# Autodesk Inventor assembly: HandRight
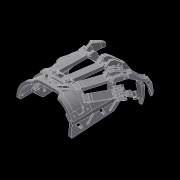
[picture p0: Inventor's stored thumbnail of the model, 180x180]
Saved by Autodesk Inventor 2015 SP1 (Build 190203100, 203)
## iProperties
Created: 2014-12-21
Part Number: HandRight
Document SubType Name: Assembly
Designer: Inventor
Mass: 48.1874 g
Surface Area: 412.068 cm^2
Volume: 48.1874 cm^3
Density: 1 g/cm^3
Author: Inventor
## Documents named in this file (22)
- E:\Exo\Models\3D\HandRight.iam
- E:\Exo\Models\3D\HandShockPlateRight.ipt
- E:\Exo\Models\3D\ThumbShockPlateRight.ipt
- E:\Exo\Models\3D\HandRibRight.ipt
- E:\Exo\Models\3D\ThumbMount.ipt
- E:\Exo\Models\3D\MetacarpusIndex.ipt
- E:\Exo\Models\3D\MetacarpusMiddle.ipt
- E:\Exo\Models\3D\MetacarpusRing.ipt
- E:\Exo\Models\3D\MetacarpusPinky.ipt
- E:\Exo\Models\3D\MetacarpusThumb.ipt
- E:\Exo\Models\3D\ProxPhalangeIndex.ipt
- E:\Exo\Models\3D\ProxPhalangeMiddle.ipt
- E:\Exo\Models\3D\ProxPhalangePinky.ipt
- E:\Exo\Models\3D\ProxPhalangeRing.ipt
- E:\Exo\Models\3D\ProxPhalangeThumb.ipt
- E:\Exo\Models\3D\Knuckle.ipt
- E:\Exo\Models\3D\KnuckleSide.ipt
- E:\Exo\Models\3D\DistPhalangeIndex.ipt
- E:\Exo\Models\3D\DistPhalangeMiddle.ipt
- E:\Exo\Models\3D\DistPhalangePinky.ipt
- E:\Exo\Models\3D\DistPhalangeRing.ipt
- E:\Exo\Models\3D\DistPhalangeThumb.ipt
## Components (34 placed, 21 different names)
1. HandShockPlateRight:1 — Mate:2, Mate:4, Mate:5, Mate:11, Mate:12, Mate:13, Mate:14
2. ThumbShockPlateRight:1 — Mate:4, Mate:5, Mate:6, Mate:7, Mate:10
3. HandRibRight:1 — Mate:2
4. ThumbMount:1 — Mate:6, Mate:7, Mate:8, Mate:9, Mate:10
5. MetacarpusIndex:1 — Mate:11, Mate:20, Mate:21, Mate:42, Mate:44, Mate:46
6. MetacarpusMiddle:1 — Mate:12, Mate:22, Mate:23, Mate:48, Mate:49, Mate:51, Mate:52
7. MetacarpusRing:1 — Mate:13, Mate:24, Mate:25, Mate:54, Mate:55, Mate:57, Mate:58
8. MetacarpusPinky:1 — Mate:14, Mate:26, Mate:27, Mate:60, Mate:61, Mate:63, Mate:64
9. MetacarpusThumb:1 — Mate:8, Mate:9, Mate:16, Mate:17, Mate:36, Mate:39
10. ProxPhalangeIndex:1 — Mate:28, Mate:29, Mate:43, Mate:45, Mate:47, Mate:66
11. ProxPhalangeMiddle:1 — Mate:30, Mate:31, Mate:50, Mate:53, Mate:67
12. ProxPhalangePinky:1 — Mate:34, Mate:35, Mate:62, Mate:65, Mate:69
13. ProxPhalangeRing:1 — Mate:32, Mate:33, Mate:56, Mate:59, Mate:68
14. ProxPhalangeThumb:1 — Mate:18, Mate:19, Mate:37, Mate:38, Mate:40, Mate:41, Mate:70
15. Knuckle:1 — Mate:26, Mate:27, Mate:34, Mate:35
16. Knuckle:2 — Mate:24, Mate:25, Mate:32, Mate:33
17. Knuckle:3 — Mate:22, Mate:23, Mate:30, Mate:31
18. Knuckle:4 — Mate:20, Mate:21, Mate:28, Mate:29
19. Knuckle:5 — Mate:16, Mate:17, Mate:18, Mate:19
20. KnuckleSide:1 — Mate:36, Mate:37, Mate:38
21. KnuckleSide:2 — Mate:39, Mate:40, Mate:41
22. KnuckleSide:3 — Mate:42, Mate:43, Mate:44
23. KnuckleSide:4 — Mate:45, Mate:46, Mate:47
24. KnuckleSide:5 — Mate:48, Mate:49, Mate:50
25. KnuckleSide:6 — Mate:51, Mate:52, Mate:53
26. KnuckleSide:7 — Mate:54, Mate:55, Mate:56
27. KnuckleSide:8 — Mate:57, Mate:58, Mate:59
28. KnuckleSide:9 — Mate:63, Mate:64, Mate:65
29. KnuckleSide:10 — Mate:60, Mate:61, Mate:62
30. DistPhalangeIndex:1 — Mate:66
31. DistPhalangeMiddle:1 — Mate:67
32. DistPhalangePinky:1 — Mate:69
33. DistPhalangeRing:1 — Mate:68
34. DistPhalangeThumb:1 — Mate:70
## Relationships (67: Mate 67)
- Mate:2: HandShockPlateRight:1 ↔ HandRibRight:1
- Mate:4: HandShockPlateRight:1 ↔ ThumbShockPlateRight:1
- Mate:5: HandShockPlateRight:1 ↔ ThumbShockPlateRight:1
- Mate:6: ThumbShockPlateRight:1 ↔ ThumbMount:1
- Mate:7: ThumbShockPlateRight:1 ↔ ThumbMount:1
- Mate:8: ThumbMount:1 ↔ MetacarpusThumb:1
- Mate:9: ThumbMount:1 ↔ MetacarpusThumb:1
- Mate:10: ThumbShockPlateRight:1 ↔ ThumbMount:1
- Mate:11: HandShockPlateRight:1 ↔ MetacarpusIndex:1
- Mate:12: HandShockPlateRight:1 ↔ MetacarpusMiddle:1
- Mate:13: HandShockPlateRight:1 ↔ MetacarpusRing:1
- Mate:14: HandShockPlateRight:1 ↔ MetacarpusPinky:1
- Mate:16: MetacarpusThumb:1 ↔ Knuckle:5
- Mate:17: MetacarpusThumb:1 ↔ Knuckle:5
- Mate:18: ProxPhalangeThumb:1 ↔ Knuckle:5
- Mate:19: ProxPhalangeThumb:1 ↔ Knuckle:5
- Mate:20: MetacarpusIndex:1 ↔ Knuckle:4
- Mate:21: MetacarpusIndex:1 ↔ Knuckle:4
- Mate:22: MetacarpusMiddle:1 ↔ Knuckle:3
- Mate:23: MetacarpusMiddle:1 ↔ Knuckle:3
- Mate:24: MetacarpusRing:1 ↔ Knuckle:2
- Mate:25: MetacarpusRing:1 ↔ Knuckle:2
- Mate:26: MetacarpusPinky:1 ↔ Knuckle:1
- Mate:27: MetacarpusPinky:1 ↔ Knuckle:1
- Mate:28: ProxPhalangeIndex:1 ↔ Knuckle:4
- Mate:29: ProxPhalangeIndex:1 ↔ Knuckle:4
- Mate:30: ProxPhalangeMiddle:1 ↔ Knuckle:3
- Mate:31: ProxPhalangeMiddle:1 ↔ Knuckle:3
- Mate:32: ProxPhalangeRing:1 ↔ Knuckle:2
- Mate:33: ProxPhalangeRing:1 ↔ Knuckle:2
- Mate:34: ProxPhalangePinky:1 ↔ Knuckle:1
- Mate:35: ProxPhalangePinky:1 ↔ Knuckle:1
- Mate:36: MetacarpusThumb:1 ↔ KnuckleSide:1
- Mate:37: ProxPhalangeThumb:1 ↔ KnuckleSide:1
- Mate:38: ProxPhalangeThumb:1 ↔ KnuckleSide:1
- Mate:39: MetacarpusThumb:1 ↔ KnuckleSide:2
- Mate:40: ProxPhalangeThumb:1 ↔ KnuckleSide:2
- Mate:41: ProxPhalangeThumb:1 ↔ KnuckleSide:2
- Mate:42: MetacarpusIndex:1 ↔ KnuckleSide:3
- Mate:43: ProxPhalangeIndex:1 ↔ KnuckleSide:3
- Mate:44: MetacarpusIndex:1 ↔ KnuckleSide:3
- Mate:45: ProxPhalangeIndex:1 ↔ KnuckleSide:4
- Mate:46: MetacarpusIndex:1 ↔ KnuckleSide:4
- Mate:47: ProxPhalangeIndex:1 ↔ KnuckleSide:4
- Mate:48: MetacarpusMiddle:1 ↔ KnuckleSide:5
- Mate:49: MetacarpusMiddle:1 ↔ KnuckleSide:5
- Mate:50: ProxPhalangeMiddle:1 ↔ KnuckleSide:5
- Mate:51: MetacarpusMiddle:1 ↔ KnuckleSide:6
- Mate:52: MetacarpusMiddle:1 ↔ KnuckleSide:6
- Mate:53: ProxPhalangeMiddle:1 ↔ KnuckleSide:6
- Mate:54: MetacarpusRing:1 ↔ KnuckleSide:7
- Mate:55: MetacarpusRing:1 ↔ KnuckleSide:7
- Mate:56: ProxPhalangeRing:1 ↔ KnuckleSide:7
- Mate:57: MetacarpusRing:1 ↔ KnuckleSide:8
- Mate:58: MetacarpusRing:1 ↔ KnuckleSide:8
- Mate:59: ProxPhalangeRing:1 ↔ KnuckleSide:8
- Mate:60: MetacarpusPinky:1 ↔ KnuckleSide:10
- Mate:61: MetacarpusPinky:1 ↔ KnuckleSide:10
- Mate:62: ProxPhalangePinky:1 ↔ KnuckleSide:10
- Mate:63: MetacarpusPinky:1 ↔ KnuckleSide:9
- Mate:64: MetacarpusPinky:1 ↔ KnuckleSide:9
- Mate:65: ProxPhalangePinky:1 ↔ KnuckleSide:9
- Mate:66: ProxPhalangeIndex:1 ↔ DistPhalangeIndex:1
- Mate:67: ProxPhalangeMiddle:1 ↔ DistPhalangeMiddle:1
- Mate:68: ProxPhalangeRing:1 ↔ DistPhalangeRing:1
- Mate:69: ProxPhalangePinky:1 ↔ DistPhalangePinky:1
- Mate:70: ProxPhalangeThumb:1 ↔ DistPhalangeThumb:1
